# Autodesk Inventor assembly: TrayAssembly
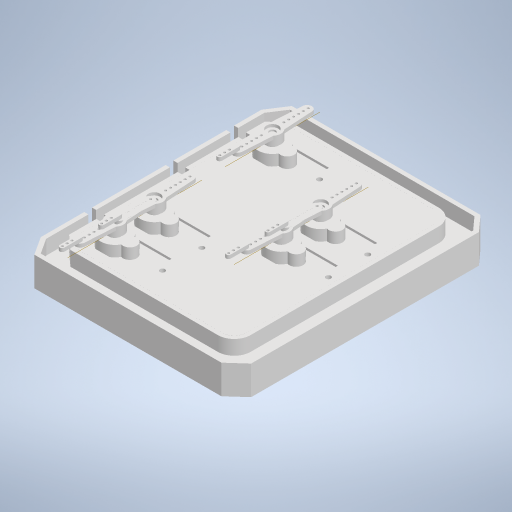
[picture p0: Inventor's stored thumbnail of the model, 512x512]
Saved by Autodesk Inventor 2023 (Build 270158000, 158)
## iProperties
Created: 2023-03-22
Part Number: TrayAssembly
Document SubType Name: Assembly
Designer: 1senadi
Author: 1senadi
## Documents named in this file (4)
- C:\Users\1senadi\Downloads\TrayAssembly.iam
- C:\Users\1senadi\Downloads\Robotic_Template_Tray.ipt
- C:\Users\1senadi\Downloads\Robotic Hand Tray.ipt
- C:\Users\1senadi\Downloads\ServoMotorAssembly.iam
## Components (7 placed, 3 different names)
1. Robotic_Template_Tray:1 — Mate:1, Mate:2
2. Robotic Hand Tray:1 — Mate:1, Mate:2, Mate:3, Mate:4, Mate:5, Mate:6, Mate:7, Mate:8, Mate:9, Mate:10, Mate:11, Mate:12
3. ServoMotorAssembly:1 [sub-assembly] — Mate:11, Mate:12
4. ServoMotorAssembly:2 [sub-assembly] — Mate:9, Mate:10
5. ServoMotorAssembly:3 [sub-assembly] — Mate:7, Mate:8
6. ServoMotorAssembly:4 [sub-assembly] — Mate:5, Mate:6
7. ServoMotorAssembly:5 [sub-assembly] — Mate:3, Mate:4
## Relationships (12: Mate 12)
- Mate:1: Robotic_Template_Tray:1 ↔ Robotic Hand Tray:1
- Mate:2: Robotic_Template_Tray:1 ↔ Robotic Hand Tray:1
- Mate:3: Robotic Hand Tray:1 ↔ ServoMotorAssembly:5
- Mate:4: Robotic Hand Tray:1 ↔ ServoMotorAssembly:5
- Mate:5: Robotic Hand Tray:1 ↔ ServoMotorAssembly:4
- Mate:6: Robotic Hand Tray:1 ↔ ServoMotorAssembly:4
- Mate:7: Robotic Hand Tray:1 ↔ ServoMotorAssembly:3
- Mate:8: Robotic Hand Tray:1 ↔ ServoMotorAssembly:3
- Mate:9: Robotic Hand Tray:1 ↔ ServoMotorAssembly:2
- Mate:10: Robotic Hand Tray:1 ↔ ServoMotorAssembly:2
- Mate:11: Robotic Hand Tray:1 ↔ ServoMotorAssembly:1
- Mate:12: Robotic Hand Tray:1 ↔ ServoMotorAssembly:1
